# Autodesk Inventor assembly: gps_holder-asm
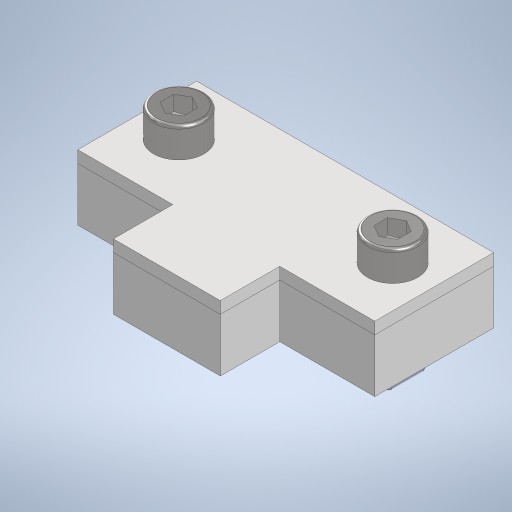
[picture p0: Inventor's stored thumbnail of the model, 512x512]
Saved by Autodesk Inventor 2024 (Build 280153000, 153)
## iProperties
Created: 2025-12-27
Part Number: gps_holder-asm
Document SubType Name: Assembly
Designer: schar
Author: schar
## Documents named in this file (5)
- C:\Users\schar\Desktop\projectBlueprint\AMSTS\hardware\gps_holder-asm.iam
- C:\Users\schar\Desktop\projectBlueprint\AMSTS\hardware\gps_holder.ipt
- C:\Users\schar\Desktop\projectBlueprint\AMSTS\hardware\gps_lid.ipt
- C:\Users\schar\Desktop\projectBlueprint\AMSTS\hardware\tnut_m5_2020.ipt
- C:\Users\schar\Documents\Inventor\Content Center Files\R2024\en-US\ISO 4762(1)\DIN EN ISO 4762 - M5 x 16.ipt
## Components (6 placed, 4 different names)
1. gps_holder:1 — Mate:1, Mate:2, Mate:3, Mate:4, Rigid:1, Rigid:2
2. gps_lid:1 — Mate:1, Mate:2, Mate:3, Mate:4, Mate:5, Mate:6
3. tnut_m5_2020:1 — Rigid:1, Mate:7
4. tnut_m5_2020:2 — Rigid:2, Mate:8
5. DIN EN ISO 4762 M5 x 16:1 — Mate:5, Mate:8
6. DIN EN ISO 4762 M5 x 16:2 — Mate:6, Mate:7
## Relationships (10: Mate 8, WeldJoint 2)
- Mate:1: gps_holder:1 ↔ gps_lid:1
- Mate:2: gps_holder:1 ↔ gps_lid:1
- Mate:3: gps_holder:1 ↔ gps_lid:1
- Mate:4: gps_holder:1 ↔ gps_lid:1
- Rigid:1 [WeldJoint] (0.159 mm): gps_holder:1 ↔ tnut_m5_2020:1
- Rigid:2 [WeldJoint] (0.159 mm): gps_holder:1 ↔ tnut_m5_2020:2
- Mate:5: gps_lid:1 ↔ DIN EN ISO 4762 M5 x 16:1
- Mate:6: gps_lid:1 ↔ DIN EN ISO 4762 M5 x 16:2
- Mate:7: tnut_m5_2020:1 ↔ DIN EN ISO 4762 M5 x 16:2
- Mate:8: tnut_m5_2020:2 ↔ DIN EN ISO 4762 M5 x 16:1
